# Autodesk Inventor assembly: 1LabKert
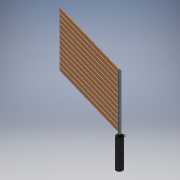
[picture p0: Inventor's stored thumbnail of the model, 180x180]
Saved by Autodesk Inventor 2019 (Build 230136000, 136)
## iProperties
Created: 2025-01-08
Part Number: 1LabKert
Document SubType Name: Assembly
Designer: laca
Mass: 115421 g
Surface Area: 180993 cm^2
Volume: 180429 cm^3
Density: 0.639701 g/cm^3
Author: laca
## Documents named in this file (4)
- C:\Users\laca\Documents\Inventor\Kerites\1LabKert.iam
- C:\Users\laca\Documents\Inventor\Kerites\L60x2profilSas.ipt
- C:\Users\laca\Documents\Inventor\Kerites\Kertdeszka.ipt
- C:\Users\laca\Documents\Inventor\Kerites\Beton.ipt
## Components (14 placed, 3 different names)
1. L60x2profilSas:1 — Mate:1, Mate:2, Insert:1, Flush:1
2. Beton:1 — Insert:1
3. Kertdeszka:1 — Mate:1, Mate:2, Flush:1
4. Kertdeszka:2
5. Kertdeszka:3
6. Kertdeszka:4
7. Kertdeszka:5
8. Kertdeszka:6
9. Kertdeszka:7
10. Kertdeszka:8
11. Kertdeszka:9
12. Kertdeszka:10
13. Kertdeszka:11
14. Kertdeszka:12
## Component patterns: (12 elements, first: Kertdeszka:1)
## Relationships (4: Mate 2, Insert 1, Flush 1)
- Mate:1: L60x2profilSas:1 ↔ Kertdeszka:1
- Mate:2: L60x2profilSas:1 ↔ Kertdeszka:1
- Insert:1: L60x2profilSas:1 ↔ Beton:1
- Flush:1: L60x2profilSas:1 ↔ Kertdeszka:1
